# Autodesk Inventor assembly: Assembly1
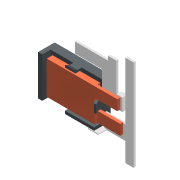
[picture p0: Inventor's stored thumbnail of the model, 180x180]
Saved by Autodesk Inventor 2021 (Build 250183000, 183)
## iProperties
Created: 2025-07-03
Part Number: Assembly1
Document SubType Name: Assembly
Designer: Owner
Author: Owner
## Documents named in this file (4)
- C:\Users\Owner\Desktop\Reza_BF23\Assembly1.iam
- C:\Users\Owner\Desktop\Reza_BF23\Catcher.ipt
- C:\Users\Owner\Desktop\Reza_BF23\TerminalL.ipt
- C:\Users\Owner\Desktop\Reza_BF23\Thermistor.ipt
## Components (3 placed, 3 different names)
1. Catcher:1 — Mate:1, Mate:2, Mate:4
2. TerminalL:1 — Mate:3, Flush:1, Flush:2
3. Thermistor:1 — Mate:1, Mate:2, Mate:3, Flush:1, Flush:2, Mate:4
## Relationships (6: Mate 4, Flush 2)
- Mate:1: Catcher:1 ↔ Thermistor:1
- Mate:2: Catcher:1 ↔ Thermistor:1
- Mate:3: TerminalL:1 ↔ Thermistor:1
- Flush:1 (-2.54 mm): TerminalL:1 ↔ Thermistor:1
- Flush:2 (-2.54 mm): TerminalL:1 ↔ Thermistor:1
- Mate:4 (0.08 mm): Catcher:1 ↔ Thermistor:1
